# Autodesk Inventor assembly: MainModule
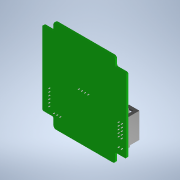
[picture p0: Inventor's stored thumbnail of the model, 180x180]
Saved by Autodesk Inventor 2021 (Build 250183000, 183)
## iProperties
Created: 2021-05-14
Part Number: MainModule
Document SubType Name: Assembly
Designer: ermoz
Author: ermoz
## Documents named in this file (14)
- D:\Moje Wyczyny\My_Poor_Projects\Sneak100_MiniSumo\minisumo-sneak100\mechanics\ElectricElements\MainModule.iam
- D:\Moje Wyczyny\My_Poor_Projects\Sneak100_MiniSumo\minisumo-sneak100\mechanics\ElectricElements\MainBoard.ipt
- D:\Moje Wyczyny\My_Poor_Projects\Sneak100_MiniSumo\minisumo-sneak100\mechanics\ElectricElements\IDC_10_pin_connector.ipt
- D:\Moje Wyczyny\My_Poor_Projects\Sneak100_MiniSumo\minisumo-sneak100\mechanics\ElectricElements\TSOP4838.ipt
- D:\Moje Wyczyny\My_Poor_Projects\Sneak100_MiniSumo\minisumo-sneak100\mechanics\ElectricElements\STM32F303RE_LQFP64.ipt
- D:\Moje Wyczyny\My_Poor_Projects\Sneak100_MiniSumo\minisumo-sneak100\mechanics\ElectricElements\SSD1306.ipt
- D:\Moje Wyczyny\My_Poor_Projects\Sneak100_MiniSumo\minisumo-sneak100\mechanics\ElectricElements\TactSwitch_6x6_8mm_SMD.ipt
- D:\Moje Wyczyny\My_Poor_Projects\Sneak100_MiniSumo\minisumo-sneak100\mechanics\ElectricElements\FemaleHeaderPin_1x6.iam
- D:\Moje Wyczyny\My_Poor_Projects\Sneak100_MiniSumo\minisumo-sneak100\mechanics\ElectricElements\Switch_ESP2010_90.ipt
- D:\Moje Wyczyny\My_Poor_Projects\Sneak100_MiniSumo\minisumo-sneak100\mechanics\ElectricElements\MaleHeaderPin_1x2.iam
- D:\Moje Wyczyny\My_Poor_Projects\Sneak100_MiniSumo\minisumo-sneak100\mechanics\ElectricElements\S9V11F5.ipt
- D:\Moje Wyczyny\My_Poor_Projects\Sneak100_MiniSumo\minisumo-sneak100\mechanics\ElectricElements\MaleHeaderPin_1x3.iam
- D:\Moje Wyczyny\My_Poor_Projects\Sneak100_MiniSumo\minisumo-sneak100\mechanics\ElectricElements\Led_0603.ipt
- D:\Moje Wyczyny\My_Poor_Projects\Sneak100_MiniSumo\minisumo-sneak100\mechanics\ElectricElements\MaleHeaderPin_1x4.iam
## Components (17 placed, 13 different names)
1. MainBoard:1 — Mate:1, Mate:3, Mate:7, Flush:1, Mate:8, Mate:9, Angle:1, Mate:17, Mate:18, Mate:19, Mate:24, Flush:4, Mate:25, Mate:26, Mate:27, Mate:29, Mate:30, Mate:31, Mate:32, Mate:34, Flush:11, Flush:12, Flush:13, Flush:14, Flush:15
2. IDC_10_pin_connector:1 — Mate:1, Flush:1, Flush:5, Flush:11
3. STM32F303RE_LQFP64:1 — Mate:3
4. TSOP4838:5 — Mate:7
5. SSD1306:1 — Mate:8, Tangent:1, Tangent:2, Tangent:3, Mate:36, Mate:37, Angle:4
6. TactSwitch_6x6_8mm_SMD:1 — Mate:17, Symmetry:1, Flush:2
7. TactSwitch_6x6_8mm_SMD:2 — Mate:18, Mate:20, Angle:3, Flush:2, Flush:3, Mate:35
8. TactSwitch_6x6_8mm_SMD:3 — Mate:19, Symmetry:1, Flush:3, Mate:34, Mate:35, Mate:36
9. FemaleHeaderPin_1x6:1 [sub-assembly] — Mate:24, Flush:13, Flush:14
10. Switch_ESP2010_90:1 — Flush:4, Mate:25, Flush:15
11. MaleHeaderPin_1x2:1 [sub-assembly] — Mate:26, Flush:5, Flush:12
12. S9V11F5:1 — Mate:28, Flush:6, Flush:7
13. MaleHeaderPin_1x3:1 [sub-assembly] — Mate:27, Mate:28, Flush:6, Flush:7
14. Led_0603:1 — Mate:29, Flush:10
15. Led_0603:2 — Mate:30, Flush:9, Flush:10
16. Led_0603:3 — Mate:31, Flush:9
17. MaleHeaderPin_1x4:1 [sub-assembly] — Mate:32, Tangent:1, Tangent:2, Tangent:3
## Relationships (47: Mate 26, Flush 14, Angle 3, Tangent 3, Symmetry 1)
- Mate:1: MainBoard:1 ↔ IDC_10_pin_connector:1
- Mate:3: MainBoard:1 ↔ STM32F303RE_LQFP64:1
- Mate:7 (3 mm): MainBoard:1 ↔ TSOP4838:5
- Flush:1: MainBoard:1 ↔ IDC_10_pin_connector:1
- Mate:8 (4 mm): MainBoard:1 ↔ SSD1306:1
- Mate:9: MainBoard:1
- Angle:1 (0 deg): MainBoard:1
- Mate:16
- Mate:17: MainBoard:1 ↔ TactSwitch_6x6_8mm_SMD:1
- Mate:18: MainBoard:1 ↔ TactSwitch_6x6_8mm_SMD:2
- Mate:19: MainBoard:1 ↔ TactSwitch_6x6_8mm_SMD:3
- Mate:20: TactSwitch_6x6_8mm_SMD:2
- Angle:3 (0 deg): TactSwitch_6x6_8mm_SMD:2
- Symmetry:1: TactSwitch_6x6_8mm_SMD:1 ↔ TactSwitch_6x6_8mm_SMD:3
- Mate:21
- Flush:2: TactSwitch_6x6_8mm_SMD:1 ↔ TactSwitch_6x6_8mm_SMD:2
- Flush:3: TactSwitch_6x6_8mm_SMD:2 ↔ TactSwitch_6x6_8mm_SMD:3
- Mate:23
- Mate:24: MainBoard:1 ↔ FemaleHeaderPin_1x6:1
- Flush:4 (1 mm): MainBoard:1 ↔ Switch_ESP2010_90:1
- Mate:25: MainBoard:1 ↔ Switch_ESP2010_90:1
- Mate:26: MainBoard:1 ↔ MaleHeaderPin_1x2:1
- Flush:5: IDC_10_pin_connector:1 ↔ MaleHeaderPin_1x2:1
- Mate:27: MainBoard:1 ↔ MaleHeaderPin_1x3:1
- Mate:28: S9V11F5:1 ↔ MaleHeaderPin_1x3:1
- Flush:6: S9V11F5:1 ↔ MaleHeaderPin_1x3:1
- Flush:7: S9V11F5:1 ↔ MaleHeaderPin_1x3:1
- Mate:29: MainBoard:1 ↔ Led_0603:1
- Mate:30: MainBoard:1 ↔ Led_0603:2
- Mate:31: MainBoard:1 ↔ Led_0603:3
- Flush:9: Led_0603:2 ↔ Led_0603:3
- Flush:10: Led_0603:1 ↔ Led_0603:2
- Mate:32: MainBoard:1 ↔ MaleHeaderPin_1x4:1
- Tangent:1 (-0.225 mm): SSD1306:1 ↔ MaleHeaderPin_1x4:1
- Tangent:2 (-0.225 mm): SSD1306:1 ↔ MaleHeaderPin_1x4:1
- Mate:34 (-7 mm): MainBoard:1 ↔ TactSwitch_6x6_8mm_SMD:3
- Tangent:3 (-0.225 mm): SSD1306:1 ↔ MaleHeaderPin_1x4:1
- Mate:35 (7 mm): TactSwitch_6x6_8mm_SMD:2 ↔ TactSwitch_6x6_8mm_SMD:3
- Flush:11 (16 mm): MainBoard:1 ↔ IDC_10_pin_connector:1
- Flush:12 (-12.5 mm): MainBoard:1 ↔ MaleHeaderPin_1x2:1
- Flush:13 (13 mm): MainBoard:1 ↔ FemaleHeaderPin_1x6:1
- Flush:14 (5 mm): MainBoard:1 ↔ FemaleHeaderPin_1x6:1
- Flush:15 (-1 mm): MainBoard:1 ↔ Switch_ESP2010_90:1
- Mate:36 (9.5 mm): SSD1306:1 ↔ TactSwitch_6x6_8mm_SMD:3
- Mate:37: SSD1306:1
- Angle:4 (0 deg): SSD1306:1
- Mate:38
